# Autodesk Inventor assembly: FrontMotorShaft
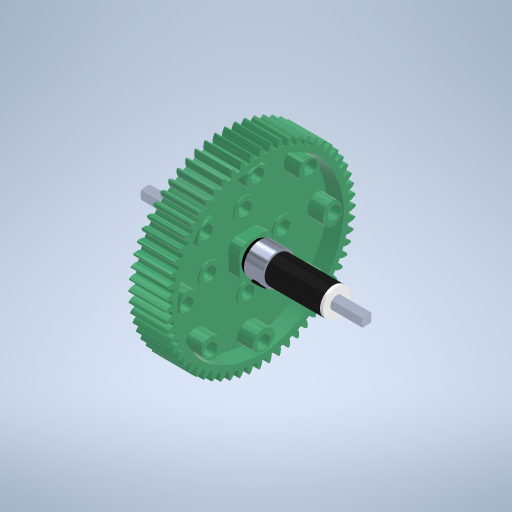
[picture p0: Inventor's stored thumbnail of the model, 512x512]
Saved by Autodesk Inventor 2023 (Build 270158000, 158)
## iProperties
Created: 2022-08-31
Part Number: FrontMotorShaft
Document SubType Name: Assembly
Designer: alex
Author: alex
## Documents named in this file (11)
- C:\Users\alex\Documents\GitHub\4067X_spin_up_cad\Chassis\FrontMotorShaft.iam
- C:\Users\alex\Documents\GitHub\4067X_spin_up_cad\Library\Motion\Spacers\Spacer Nylon .375 OD\NSpacer .375 OD x .125.ipt
- C:\Users\alex\Documents\GitHub\4067X_spin_up_cad\Library\Motion\Spacers\Spacer Nylon .375 OD.ipt
- C:\Users\alex\Documents\GitHub\4067X_spin_up_cad\Library\Motion\Gears\HS 60T Gear, Square.ipt
- C:\Users\alex\Documents\GitHub\4067X_spin_up_cad\Library\Motion\Shaft Collar with Set Screw.ipt
- C:\Users\alex\Documents\GitHub\4067X_spin_up_cad\Library\Motion\Spacers\Spacer Nylon .375 OD\NSpacer .375 OD x .500.ipt
- C:\Users\alex\Documents\GitHub\4067X_spin_up_cad\Library\Motion\Spacers\Washer Teflon\TWasher .375 OD x .04000.ipt
- C:\Users\alex\Documents\GitHub\4067X_spin_up_cad\Library\Motion\Spacers\Washer Teflon.ipt
- C:\Users\alex\Documents\GitHub\4067X_spin_up_cad\Library\Motion\Spacers\Spacer Nylon .375 OD\NSpacer .375 OD x .250.ipt
- C:\Users\alex\Documents\GitHub\4067X_spin_up_cad\Library\Motion\Shaft LS.ipt
- C:\Users\alex\Documents\GitHub\4067X_spin_up_cad\Library\Motion\Shaft LS\Shaft LS 3.0 in.ipt
## Components (7 placed, 7 different names)
1. NSpacer .375 OD x .125:1 — Insert:1, Flush:1
2. HS 60T Gear, Square:1 — Insert:1, Insert:2, Mate:1, Mate:2
3. Shaft Collar with Set Screw:1 — Insert:2, Insert:3
4. NSpacer .375 OD x .500:2 — Insert:3, Insert:4
5. NSpacer .375 OD x .250:3 — Insert:4, Insert:5
6. TWasher .375 OD x .04000:1 — Insert:5
7. Shaft LS 3.0 in:1 — Mate:1, Mate:2, Flush:1
## Relationships (8: Insert 5, Mate 2, Flush 1)
- Insert:1: NSpacer .375 OD x .125:1 ↔ HS 60T Gear, Square:1
- Insert:2: HS 60T Gear, Square:1 ↔ Shaft Collar with Set Screw:1
- Insert:3: Shaft Collar with Set Screw:1 ↔ NSpacer .375 OD x .500:2
- Insert:4: NSpacer .375 OD x .500:2 ↔ NSpacer .375 OD x .250:3
- Insert:5: NSpacer .375 OD x .250:3 ↔ TWasher .375 OD x .04000:1
- Mate:1: HS 60T Gear, Square:1 ↔ Shaft LS 3.0 in:1
- Mate:2: HS 60T Gear, Square:1 ↔ Shaft LS 3.0 in:1
- Flush:1 (24.003 mm): NSpacer .375 OD x .125:1 ↔ Shaft LS 3.0 in:1
